# Autodesk Inventor assembly: 7inDisplayAssembly
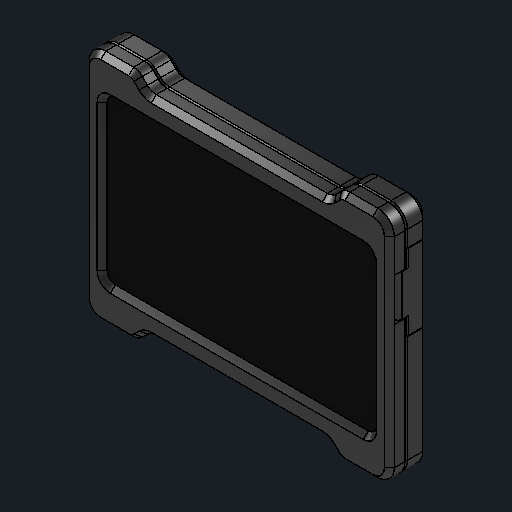
[picture p0: Inventor's stored thumbnail of the model, 512x512]
Saved by Autodesk Inventor 2026.2 (Build 302298000, 298)
## iProperties
Created: 2026-01-24
Part Number: 7inDisplayAssembly
Document SubType Name: Assembly
Designer: JoshuaEah
Author: JoshuaEah
## Documents named in this file (7)
- C:\Users\JoshuaEah\Documents\GitHub\Designed-Trinkets\7in Touch Display\7inDisplayAssembly.iam
- C:\Users\JoshuaEah\Documents\GitHub\Designed-Trinkets\7in Touch Display\Parts\7in Display Module.iam
- C:\Users\JoshuaEah\Documents\GitHub\Designed-Trinkets\7in Touch Display\Parts\7in Touch Display Faceplate.ipt
- C:\Users\JoshuaEah\Documents\GitHub\Designed-Trinkets\7in Touch Display\Parts\Hardware\M3 Threaded Insert.ipt
- C:\Users\JoshuaEah\Documents\GitHub\Designed-Trinkets\7in Touch Display\Parts\7in Touch Display Backplate.ipt
- C:\Users\JoshuaEah\Documents\GitHub\Designed-Trinkets\7in Touch Display\Parts\Hardware\M3x14 SHCS.ipt
- C:\Users\JoshuaEah\Documents\GitHub\Designed-Trinkets\7in Touch Display\Parts\7in Touch Display IO Cover.ipt
## Components (12 placed, 6 different names)
1. 7in Display Module:1 [sub-assembly] — Insert:1, Insert:2
2. 7in Touch Display Faceplate:1 — Insert:1, Insert:2, Insert:3, Insert:4, Insert:5, Insert:6, Mate:1, Mate:2, Mate:3, Rotational:1
3. 7in Touch Display Backplate:1 — Mate:1, Mate:2, Mate:3, Insert:7, Insert:8, Insert:9, Insert:10
4. 7in Touch Display IO Cover:1 — Rotational:1
5. M3 Threaded Insert:1 — Insert:3
6. M3 Threaded Insert:2 — Insert:4
7. M3 Threaded Insert:3 — Insert:6
8. M3 Threaded Insert:4 — Insert:5
9. M3x14 SHCS:1 — Insert:7
10. M3x14 SHCS:2 — Insert:8
11. M3x14 SHCS:3 — Insert:9
12. M3x14 SHCS:4 — Insert:10
## Relationships (14: Insert 10, Mate 3, RevoluteJoint 1)
- Insert:1: 7in Display Module:1 ↔ 7in Touch Display Faceplate:1
- Insert:2: 7in Display Module:1 ↔ 7in Touch Display Faceplate:1
- Insert:3: 7in Touch Display Faceplate:1 ↔ M3 Threaded Insert:1
- Insert:4: 7in Touch Display Faceplate:1 ↔ M3 Threaded Insert:2
- Insert:5: 7in Touch Display Faceplate:1 ↔ M3 Threaded Insert:4
- Insert:6: 7in Touch Display Faceplate:1 ↔ M3 Threaded Insert:3
- Mate:1: 7in Touch Display Faceplate:1 ↔ 7in Touch Display Backplate:1
- Mate:2: 7in Touch Display Faceplate:1 ↔ 7in Touch Display Backplate:1
- Mate:3: 7in Touch Display Faceplate:1 ↔ 7in Touch Display Backplate:1
- Insert:7: 7in Touch Display Backplate:1 ↔ M3x14 SHCS:1
- Insert:8: 7in Touch Display Backplate:1 ↔ M3x14 SHCS:2
- Insert:9: 7in Touch Display Backplate:1 ↔ M3x14 SHCS:3
- Insert:10: 7in Touch Display Backplate:1 ↔ M3x14 SHCS:4
- Rotational:1 [RevoluteJoint] (-0.4 mm): 7in Touch Display Faceplate:1 ↔ 7in Touch Display IO Cover:1
